# Autodesk Inventor assembly: XM430_ASM_WITHOUT-BACK
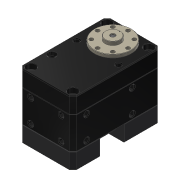
[picture p0: Inventor's stored thumbnail of the model, 180x180]
Saved by Autodesk Inventor 2019.4 (Build 234330000, 330)
## iProperties
Created: 2019-10-08
Part Number: XM430_ASM_WITHOUT-BACK
Material: 一般
Document SubType Name: Assembly
Designer: y6tada
Author: y6tada
## Documents named in this file (5)
- C:\Workspace\Yuni9\Inventor\Libs\DYNAMIXEL\XM430\XM430_ASM_WITHOUT-BACK.iam
- C:\Workspace\Yuni9\Inventor\Libs\DYNAMIXEL\XM430\XM430_HOUSING_MIDDLE.ipt
- C:\Workspace\Yuni9\Inventor\Libs\DYNAMIXEL\XM430\XM430_HOUSING_TOP.ipt
- C:\Workspace\Yuni9\Inventor\Libs\DYNAMIXEL\XM430\XM430_HORN.ipt
- C:\Workspace\Yuni9\Inventor\Libs\DYNAMIXEL\XM430\XM430_HOUSING_BOTTOM.ipt
## Components (4 placed, 4 different names)
1. XM430_HOUSING_MIDDLE:1 — フラッシュ:1, フラッシュ:2, フラッシュ:3, フラッシュ:4, フラッシュ:5, メイト:1, フラッシュ:7
2. XM430_HOUSING_TOP:1 — フラッシュ:4, フラッシュ:5, メイト:1, メイト:2, メイト:3, フラッシュ:6
3. XM430_HORN:1 — メイト:2, メイト:3, フラッシュ:6
4. XM430_HOUSING_BOTTOM:1 — フラッシュ:7, メイト:9, フラッシュ:8
## Relationships (12: Flush 8, Mate 4)
- フラッシュ:1 [Flush]: XM430_HOUSING_MIDDLE:1
- フラッシュ:2 [Flush]: XM430_HOUSING_MIDDLE:1
- フラッシュ:3 [Flush]: XM430_HOUSING_MIDDLE:1
- フラッシュ:4 [Flush]: XM430_HOUSING_MIDDLE:1 ↔ XM430_HOUSING_TOP:1
- フラッシュ:5 [Flush]: XM430_HOUSING_MIDDLE:1 ↔ XM430_HOUSING_TOP:1
- メイト:1 [Mate]: XM430_HOUSING_MIDDLE:1 ↔ XM430_HOUSING_TOP:1
- メイト:2 [Mate]: XM430_HOUSING_TOP:1 ↔ XM430_HORN:1
- メイト:3 [Mate]: XM430_HOUSING_TOP:1 ↔ XM430_HORN:1
- フラッシュ:6 [Flush]: XM430_HOUSING_TOP:1 ↔ XM430_HORN:1
- フラッシュ:7 [Flush]: XM430_HOUSING_MIDDLE:1 ↔ XM430_HOUSING_BOTTOM:1
- メイト:9 [Mate]: XM430_HOUSING_BOTTOM:1
- フラッシュ:8 [Flush]: XM430_HOUSING_BOTTOM:1
